# Autodesk Inventor assembly: Assembly2
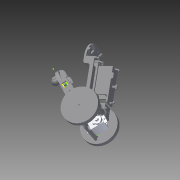
[picture p0: Inventor's stored thumbnail of the model, 180x180]
Saved by Autodesk Inventor 2015 (Build 190159000, 159)
## iProperties
Created: 2014-12-09
Part Number: Assembly2
Document SubType Name: Assembly
Designer: Temp2
Author: Temp2
## Documents named in this file (13)
- C:\Users\JT\Desktop\Thesis\LaTeX\Thesis\CD\Prototype 1\Assembly2.iam
- C:\Users\JT\Desktop\Thesis\LaTeX\Thesis\CD\Prototype 1\Motor_Enclosure.ipt
- C:\Users\JT\Desktop\Thesis\LaTeX\Thesis\CD\Prototype 1\Models\Pivot_Rod.ipt
- C:\Users\JT\Desktop\Thesis\LaTeX\Thesis\CD\Prototype 1\Top_Platform_Extended.ipt
- C:\Users\JT\Desktop\Thesis\LaTeX\Thesis\CD\Prototype 1\Models\HD-1900A_Servo.ipt
- C:\Users\JT\Desktop\Thesis\LaTeX\Thesis\CD\Prototype 1\Models\Motor_Bracket.ipt
- C:\Users\JT\Desktop\Thesis\LaTeX\Thesis\CD\Prototype 1\Models\Motors.ipt
- C:\Users\JT\Desktop\Thesis\LaTeX\Thesis\CD\Prototype 1\Component_Clip_A.ipt
- C:\Users\JT\Desktop\Thesis\LaTeX\Thesis\CD\Prototype 1\Models\Caster.ipt
- C:\Users\JT\Desktop\Thesis\LaTeX\Thesis\CD\Prototype 1\Models\Power_Switch.ipt
- C:\Users\JT\Desktop\Thesis\LaTeX\Thesis\CD\Prototype 1\Models\Power_Socket.ipt
- C:\Users\JT\Desktop\Thesis\LaTeX\Thesis\CD\Prototype 1\Base_Platform_Extended_Model2.1.ipt
- C:\Users\JT\Desktop\Thesis\LaTeX\Thesis\CD\Rattus_Parts\Models\Wheel.ipt
## Components (15 placed, 12 different names)
1. Motor_Enclosure:1 — Mate:4, Mate:7, Mate:15, Mate:36, Mate:37, Mate:38
2. Pivot_Rod:1 — Mate:4, Mate:5, Mate:8
3. Top_Platform_Extended:1 — Mate:5, Mate:8, Mate:17, Mate:23, Mate:24, Flush:5
4. HD-1900A_Servo:1 — Mate:7, Mate:15, Mate:39
5. Motor_Bracket:1 — Mate:12, Mate:13, Mate:14, Mate:27, Mate:28, Mate:29
6. Motors:1 — Mate:12, Mate:13, Mate:14, Mate:45, Mate:46
7. Component_Clip_A:1 — Mate:17, Mate:23, Mate:24
8. Caster:1 — Mate:33, Mate:34, Mate:35
9. Power_Switch:1 — Mate:40, Flush:6, Mate:41, Mate:42
10. Power_Socket:1 — Mate:43, Mate:44
11. Motors:2 — Flush:4, Mate:25, Mate:26, Mate:30, Mate:32, Mate:47, Mate:48
12. Motor_Bracket:2 — Flush:4, Mate:25, Mate:26, Mate:31, Flush:5
13. Base_Platform_Extended_Model2.1:1 — Mate:27, Mate:28, Mate:29, Mate:30, Mate:31, Mate:32, Mate:33, Mate:34, Mate:35, Mate:36, Mate:37, Mate:38, Mate:39, Mate:40, Flush:6, Mate:41, Mate:42, Mate:43, Mate:44
14. Wheel:1 — Mate:45, Mate:46
15. Wheel:2 — Mate:47, Mate:48
## Relationships (38: Mate 35, Flush 3)
- Mate:4: Motor_Enclosure:1 ↔ Pivot_Rod:1
- Mate:5: Pivot_Rod:1 ↔ Top_Platform_Extended:1
- Mate:7: Motor_Enclosure:1 ↔ HD-1900A_Servo:1
- Mate:8: Pivot_Rod:1 ↔ Top_Platform_Extended:1
- Mate:12: Motor_Bracket:1 ↔ Motors:1
- Mate:13: Motor_Bracket:1 ↔ Motors:1
- Mate:14: Motor_Bracket:1 ↔ Motors:1
- Mate:15: Motor_Enclosure:1 ↔ HD-1900A_Servo:1
- Mate:17: Top_Platform_Extended:1 ↔ Component_Clip_A:1
- Mate:23: Top_Platform_Extended:1 ↔ Component_Clip_A:1
- Mate:24: Top_Platform_Extended:1 ↔ Component_Clip_A:1
- Flush:4: Motors:2 ↔ Motor_Bracket:2
- Mate:25: Motors:2 ↔ Motor_Bracket:2
- Mate:26: Motors:2 ↔ Motor_Bracket:2
- Mate:27: Motor_Bracket:1 ↔ Base_Platform_Extended_Model2.1:1
- Mate:28: Motor_Bracket:1 ↔ Base_Platform_Extended_Model2.1:1
- Mate:29: Motor_Bracket:1 ↔ Base_Platform_Extended_Model2.1:1
- Mate:30: Motors:2 ↔ Base_Platform_Extended_Model2.1:1
- Mate:31: Motor_Bracket:2 ↔ Base_Platform_Extended_Model2.1:1
- Mate:32: Motors:2 ↔ Base_Platform_Extended_Model2.1:1
- Mate:33: Caster:1 ↔ Base_Platform_Extended_Model2.1:1
- Mate:34: Caster:1 ↔ Base_Platform_Extended_Model2.1:1
- Mate:35: Caster:1 ↔ Base_Platform_Extended_Model2.1:1
- Mate:36: Motor_Enclosure:1 ↔ Base_Platform_Extended_Model2.1:1
- Mate:37: Motor_Enclosure:1 ↔ Base_Platform_Extended_Model2.1:1
- Mate:38: Motor_Enclosure:1 ↔ Base_Platform_Extended_Model2.1:1
- Flush:5: Top_Platform_Extended:1 ↔ Motor_Bracket:2
- Mate:39: HD-1900A_Servo:1 ↔ Base_Platform_Extended_Model2.1:1
- Mate:40: Power_Switch:1 ↔ Base_Platform_Extended_Model2.1:1
- Flush:6: Power_Switch:1 ↔ Base_Platform_Extended_Model2.1:1
- Mate:41: Power_Switch:1 ↔ Base_Platform_Extended_Model2.1:1
- Mate:42: Power_Switch:1 ↔ Base_Platform_Extended_Model2.1:1
- Mate:43: Power_Socket:1 ↔ Base_Platform_Extended_Model2.1:1
- Mate:44: Power_Socket:1 ↔ Base_Platform_Extended_Model2.1:1
- Mate:45: Motors:1 ↔ Wheel:1
- Mate:46: Motors:1 ↔ Wheel:1
- Mate:47: Motors:2 ↔ Wheel:2
- Mate:48: Motors:2 ↔ Wheel:2
